# Autodesk Inventor assembly: BackPlate
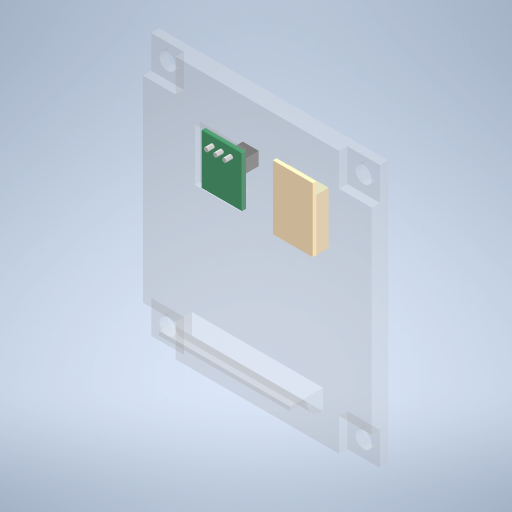
[picture p0: Inventor's stored thumbnail of the model, 512x512]
Saved by Autodesk Inventor 2023 (Build 270158000, 158)
## iProperties
Created: 2023-10-14
Part Number: BackPlate
Document SubType Name: Assembly
Designer: Gage
Author: Gage
## Documents named in this file (4)
- C:\Users\Gage\OneDrive\Desktop\Autodesk Inventor\207\BackPlate.iam
- C:\Users\Gage\OneDrive\Desktop\Autodesk Inventor\207\BackPannel.ipt
- C:\Users\Gage\OneDrive\Desktop\Autodesk Inventor\207\DHT22.ipt
- C:\Users\Gage\OneDrive\Desktop\Autodesk Inventor\207\IF Remote reader.ipt
## Components (3 placed, 3 different names)
1. BackPannel:1 — Mate:1, Mate:2, Mate:3, Mate:4
2. DHT22:1 — Mate:1, Mate:2
3. IF Remote reader:1 — Mate:3, Mate:4
## Relationships (4: Mate 4)
- Mate:1: BackPannel:1 ↔ DHT22:1
- Mate:2: BackPannel:1 ↔ DHT22:1
- Mate:3: BackPannel:1 ↔ IF Remote reader:1
- Mate:4: BackPannel:1 ↔ IF Remote reader:1
